# Autodesk Inventor assembly: arm
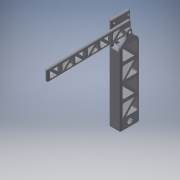
[picture p0: Inventor's stored thumbnail of the model, 180x180]
Saved by Autodesk Inventor 2019 (Build 230136000, 136)
## iProperties
Created: 2019-03-05
Part Number: arm
Document SubType Name: Assembly
Designer: s-4036947
Author: s-4036947
## Documents named in this file (4)
- \\shares\studenthome\S-4036947\Inventor Files\fbd-arm\cad\arm.iam
- \\shares\studenthome\S-4036947\Inventor Files\fbd-arm\cad\upper arm.ipt
- \\shares\studenthome\S-4036947\Inventor Files\fbd-arm\cad\Nema17.ipt
- \\shares\studenthome\S-4036947\Inventor Files\fbd-arm\cad\fore arm.ipt
## Components (3 placed, 3 different names)
1. upper arm:1 — Mate:1, Mate:6, Mate:7, Mate:8
2. Nema17:1 — Mate:1, Mate:6, Mate:7, Mate:9
3. fore arm:1 — Mate:8, Mate:9
## Relationships (5: Mate 5)
- Mate:1: upper arm:1 ↔ Nema17:1
- Mate:6: upper arm:1 ↔ Nema17:1
- Mate:7: upper arm:1 ↔ Nema17:1
- Mate:8 (3.175 mm): upper arm:1 ↔ fore arm:1
- Mate:9: Nema17:1 ↔ fore arm:1
